# Autodesk Inventor assembly: Hand Custom Gussets
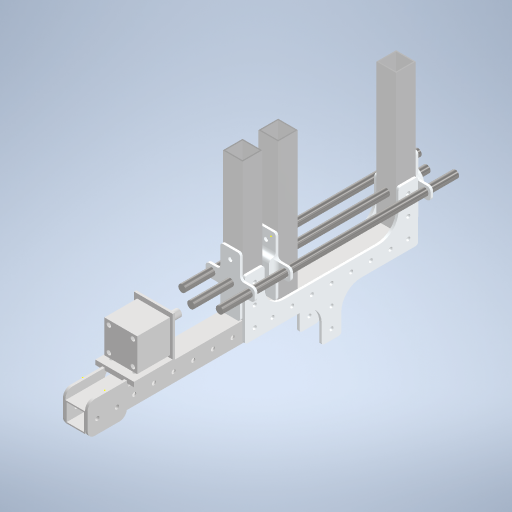
[picture p0: Inventor's stored thumbnail of the model, 512x512]
Saved by Autodesk Inventor 2024 (Build 280153000, 153)
## iProperties
Created: 2024-01-20
Part Number: Hand Custom Gussets
Document SubType Name: Assembly
Designer: aidan
Author: aidan
## Documents named in this file (12)
- C:\Users\aidan\OneDrive\Documents\Inventor\Content Center Files\Hand Custom Gussets.iam
- C:\Users\aidan\OneDrive\Documents\Inventor\Content Center Files\Tube Finger.ipt
- C:\Users\aidan\OneDrive\Documents\Inventor\Content Center Files\Lead Nut Holder Mk2.ipt
- C:\Users\aidan\OneDrive\Documents\Inventor\Content Center Files\Guide Rod Holder.ipt
- C:\Users\aidan\OneDrive\Documents\Inventor\Content Center Files\Finger Base.ipt
- C:\Users\aidan\OneDrive\Documents\Inventor\Content Center Files\Lead_Shaft.ipt
- C:\Users\aidan\OneDrive\Documents\Inventor\Content Center Files\Nema 3 Mounting.ipt
- C:\Users\aidan\OneDrive\Documents\Inventor\Content Center Files\Nema 17.ipt
- C:\Users\aidan\OneDrive\Documents\Inventor\Content Center Files\Motor Mount.ipt
- C:\Users\aidan\OneDrive\Documents\Inventor\Content Center Files\Bearing Holder.ipt
- C:\Users\aidan\OneDrive\Documents\Inventor\Content Center Files\Shaft Adapter.ipt
- C:\Users\aidan\OneDrive\Documents\Inventor\Content Center Files\Specialty Arm Gusset.ipt
## Components (16 placed, 11 different names)
1. Tube Finger:1 — Mate:1, Rotational:12
2. Tube Finger:2 — Mate:1
3. Lead Nut Holder Mk2:1
4. Tube Finger:3 — Rotational:7
5. Finger Base:1 — Rotational:14, Rotational:17, Rotational:18
6. Guide Rod Holder:2 — Rotational:7, Rotational:8, Rotational:9, Rotational:10
7. Lead_Shaft:1 — Rotational:10
8. Lead_Shaft:2 — Rotational:9
9. Lead_Shaft:3 — Rotational:8
10. Nema 3 Mounting:1 — Rotational:15
11. Nema 17:1 — Rotational:16
12. Motor Mount:1 — Rotational:14, Rotational:15
13. Bearing Holder:1 — Rotational:12
14. Shaft Adapter:1 — Rotational:16
15. Specialty Arm Gusset:1 — Rotational:18
16. Specialty Arm Gusset:2 — Rotational:17
## Relationships (11: RevoluteJoint 10, Mate 1)
- Mate:1 (127 mm): Tube Finger:1 ↔ Tube Finger:2
- Rotational:7 [RevoluteJoint]: Tube Finger:3 ↔ Guide Rod Holder:2
- Rotational:8 [RevoluteJoint] (-38.1 mm): Guide Rod Holder:2 ↔ Lead_Shaft:3
- Rotational:9 [RevoluteJoint] (-50.8 mm): Guide Rod Holder:2 ↔ Lead_Shaft:2
- Rotational:10 [RevoluteJoint] (-38.1 mm): Guide Rod Holder:2 ↔ Lead_Shaft:1
- Rotational:12 [RevoluteJoint]: Tube Finger:1 ↔ Bearing Holder:1
- Rotational:14 [RevoluteJoint]: Finger Base:1 ↔ Motor Mount:1
- Rotational:15 [RevoluteJoint]: Nema 3 Mounting:1 ↔ Motor Mount:1
- Rotational:16 [RevoluteJoint] (-6.35 mm): Nema 17:1 ↔ Shaft Adapter:1
- Rotational:17 [RevoluteJoint]: Finger Base:1 ↔ Specialty Arm Gusset:2
- Rotational:18 [RevoluteJoint]: Finger Base:1 ↔ Specialty Arm Gusset:1
